# Autodesk Inventor assembly: gantry_frame
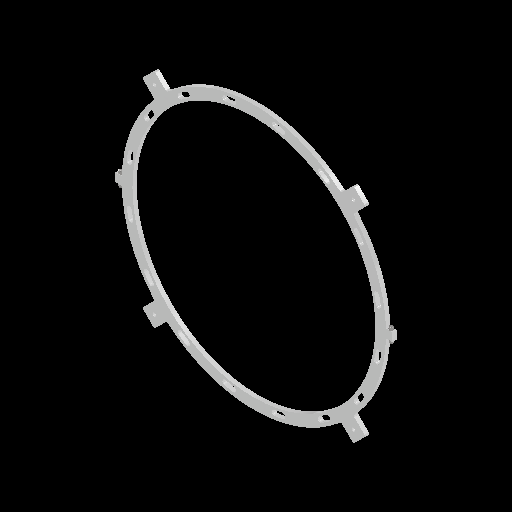
[picture p0: Inventor's stored thumbnail of the model, 512x512]
Saved by Autodesk Inventor 2026.1 (Build 301233000, 233)
## iProperties
Created: 2025-09-18
Part Number: gantry_frame
Document SubType Name: Assembly
Designer: drago
Author: drago
## Documents named in this file (5)
- C:\Users\drago\Desktop\_QIST4500_Multidisciplinary_Team_Project\Proteox MX magnet positioner CAD\gantry_frame\full_ring.iam
- C:\Users\drago\Desktop\_QIST4500_Multidisciplinary_Team_Project\Proteox MX magnet positioner CAD\gantry_frame\half_ring.ipt
- C:\Users\drago\Documents\Inventor\Content Center Files\R2026\en-US\ISO 7089\ISO 7089 - 5 - 140 HV(1).ipt
- C:\Users\drago\Documents\Inventor\Content Center Files\R2026\en-US\ISO 4762(2)\ISO 4762 - M5 x 30ISO.ipt
- C:\Users\drago\Documents\Inventor\Content Center Files\R2026\en-US\ISO 4032(2)\ISO 4032 - M5 - ISO.ipt
## Components (10 placed, 4 different names)
1. half_ring:1 — Mate:1, Mate:2, Mate:5, Mate:6, Mate:7, Mate:9, Mate:10, Mate:11
2. half_ring:2 — Mate:3, Mate:4, Mate:8, Mate:12
3. ISO 7089 5:1 — Mate:5, Mate:6, Insert:1
4. ISO 4762 M5 x 30:1 — Insert:1
5. ISO 7089 5:2 — Mate:7, Mate:8, Insert:2
6. ISO 4032 M5:1 — Insert:2
7. ISO 7089 5:3 — Mate:9, Mate:10, Insert:3
8. ISO 4762 M5 x 30:2 — Insert:3
9. ISO 7089 5:4 — Mate:11, Mate:12, Insert:4
10. ISO 4032 M5:2 — Insert:4
## Relationships (16: Mate 12, Insert 4)
- Mate:1: half_ring:1
- Mate:2: half_ring:1
- Mate:3: half_ring:2
- Mate:4: half_ring:2
- Mate:5: half_ring:1 ↔ ISO 7089 5:1
- Mate:6: half_ring:1 ↔ ISO 7089 5:1
- Insert:1: ISO 7089 5:1 ↔ ISO 4762 M5 x 30:1
- Mate:7: half_ring:1 ↔ ISO 7089 5:2
- Mate:8: half_ring:2 ↔ ISO 7089 5:2
- Insert:2: ISO 7089 5:2 ↔ ISO 4032 M5:1
- Mate:9: half_ring:1 ↔ ISO 7089 5:3
- Mate:10: half_ring:1 ↔ ISO 7089 5:3
- Insert:3: ISO 7089 5:3 ↔ ISO 4762 M5 x 30:2
- Mate:11: half_ring:1 ↔ ISO 7089 5:4
- Mate:12: half_ring:2 ↔ ISO 7089 5:4
- Insert:4: ISO 7089 5:4 ↔ ISO 4032 M5:2
